# Autodesk Inventor assembly: MAIN
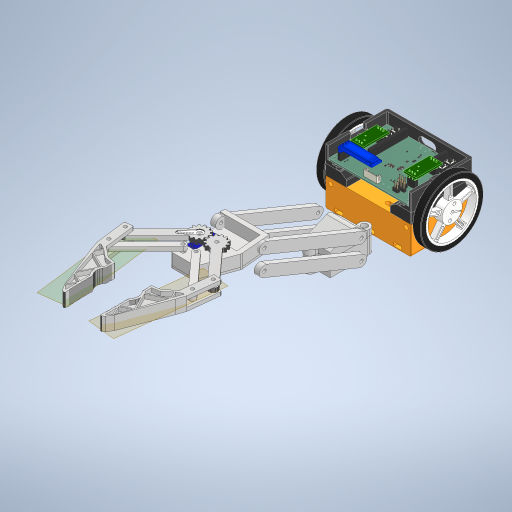
[picture p0: Inventor's stored thumbnail of the model, 512x512]
Saved by Autodesk Inventor 2023 (Build 270158000, 158)
## iProperties
Created: 2024-04-25
Part Number: MAIN
Document SubType Name: Assembly
Designer: Kamil
Author: Kamil
## Documents named in this file (24)
- C:\Users\kamil\Documents\PROJECTS - repos\ModBot---Projekt-Zespolowy\mechanics\MAIN.iam
- C:\Users\kamil\Documents\PROJECTS - repos\ModBot---Projekt-Zespolowy\mechanics\PololuWheel 60x8mm.ipt
- C:\Users\kamil\Documents\PROJECTS - repos\ModBot---Projekt-Zespolowy\mechanics\N20 DC MOTOR.ipt
- C:\Users\kamil\Documents\PROJECTS - repos\ModBot---Projekt-Zespolowy\mechanics\podst.ipt
- C:\Users\kamil\Documents\PROJECTS - repos\ModBot---Projekt-Zespolowy\mechanics\Li_Pol 800mAh.ipt
- C:\Users\kamil\Documents\PROJECTS - repos\ModBot---Projekt-Zespolowy\mechanics\pokrywka_baterii.ipt
- C:\Users\kamil\Documents\PROJECTS - repos\ModBot---Projekt-Zespolowy\mechanics\N20_Bracket_Extended_Pololu.ipt
- C:\Users\kamil\Documents\PROJECTS - repos\ModBot---Projekt-Zespolowy\mechanics\N20_Bracket_Extended_Pololu_MIR.ipt
- C:\Users\kamil\Documents\PROJECTS - repos\ModBot---Projekt-Zespolowy\mechanics\tyl.ipt
- C:\Users\kamil\Documents\PROJECTS - repos\ModBot---Projekt-Zespolowy\mechanics\podstawa_PCB.ipt
- C:\Users\kamil\Documents\PROJECTS - repos\ModBot---Projekt-Zespolowy\mechanics\pcb_glowne.ipt
- C:\Users\kamil\Documents\PROJECTS - repos\ModBot---Projekt-Zespolowy\mechanics\dach.ipt
- C:\Users\kamil\Documents\PROJECTS - repos\ModBot---Projekt-Zespolowy\mechanics\MS_podstawa.ipt
- C:\Users\kamil\Documents\PROJECTS - repos\ModBot---Projekt-Zespolowy\mechanics\TOF_VL53L0X (1).ipt
- C:\Users\kamil\Documents\PROJECTS - repos\ModBot---Projekt-Zespolowy\mechanics\MS_Pokrywa.ipt
- C:\Users\kamil\Documents\PROJECTS - repos\ModBot---Projekt-Zespolowy\mechanics\TOF_golpins.iam
- C:\Users\kamil\Documents\PROJECTS - repos\ModBot---Projekt-Zespolowy\mechanics\MS_PCB.ipt
- C:\Users\kamil\Documents\PROJECTS - repos\ModBot---Projekt-Zespolowy\mechanics\TOF_golpins_MIR.iam
- C:\Users\kamil\Documents\PROJECTS - repos\ModBot---Projekt-Zespolowy\mechanics\STEP\Płytka główna.ipt
- C:\Users\kamil\Documents\PROJECTS - repos\ModBot---Projekt-Zespolowy\mechanics\STEP\ESP32.ipt
- C:\Users\kamil\Documents\PROJECTS - repos\ModBot---Projekt-Zespolowy\mechanics\STEP\Sterowniki silników.ipt
- C:\Users\kamil\Documents\PROJECTS - repos\ModBot---Projekt-Zespolowy\mechanics\STEP\TFT Display 0.69_96x16.ipt
- C:\Users\kamil\Documents\PROJECTS - repos\ModBot---Projekt-Zespolowy\mechanics\modbot.ipt
- C:\Users\kamil\Documents\PROJECTS - repos\ModBot---Projekt-Zespolowy\mechanics\modul_chwytaka\chwytak.iam
## Components (29 placed, 23 different names)
1. PololuWheel 60x8mm:1 — Zestawiające:1, Kątowe:1, Zestawiające:2, Zestawiające:5, Zestawiające:6, Równoległe:2
2. N20 DC MOTOR:1 — Zestawiające:1, Kątowe:1, Zestawiające:2, Równoległe:1, Zestawiające:9, Zestawiające:18, Zestawiające:19
3. PololuWheel 60x8mm:2 — Zestawiające:5, Zestawiające:6, Zestawiające:10
4. N20 DC MOTOR:2 — Równoległe:1, Zestawiające:7
5. podst:1 — Zestawiające:9, Zestawiające:10, Zestawiające:11, Zestawiające:13, Równoległe:6, Zestawiające:14, Zestawiające:20, Zestawiające:33, Równoległe:22, Równoległe:23, Zestawiające:40, Zestawiające:50, Zestawiające:57, Równoległe:38
6. Li_Pol 800mAh:1 — Zestawiające:11, Zestawiające:13
7. pokrywka_baterii:1 — Równoległe:6, Zestawiające:14
8. N20_Bracket_Extended_Pololu:1 — Zestawiające:18, Zestawiające:19, Zestawiające:29, Zestawiające:69, Równoległe:37
9. N20_Bracket_Extended_Pololu_MIR:1 — Równoległe:17, Równoległe:18
10. tyl:1 — Zestawiające:20
11. podstawa_PCB:1 — Zestawiające:29, Równoległe:17, Równoległe:18, Zestawiające:30, Zestawiające:31, Równoległe:19, Równoległe:25, Zestawiające:61, Zestawiające:62, Zestawiające:63, Równoległe:35, Równoległe:36, Zestawiające:68, Zestawiające:70
12. pcb_glowne:1 — Zestawiające:30, Zestawiające:31, Równoległe:19
13. dach:1 — Równoległe:35, Równoległe:36, Zestawiające:68
14. MS_podstawa:1 — Zestawiające:33, Równoległe:22, Równoległe:23, Zestawiające:34, Zestawiające:35, Równoległe:24, Zestawiające:39, Zestawiające:43, Zestawiające:49, Zestawiające:51, Zestawiające:52, Zestawiające:56
15. TOF_VL53L0X (1):2 — Zestawiające:39, Zestawiające:40, Zestawiające:46
16. MS_Pokrywa:1 — Zestawiające:34, Zestawiające:35, Równoległe:24, Zestawiające:59
17. TOF_VL53L0X (1):4 — Zestawiające:43, Zestawiające:46
18. TOF_golpins:1 [sub-assembly] — Zestawiające:49, Zestawiające:50, Zestawiające:51, Zestawiające:54
19. TOF_golpins:2 [sub-assembly] — Zestawiające:52, Zestawiające:54, Zestawiające:58, Zestawiające:59
20. MS_PCB:1 — Zestawiające:56, Zestawiające:57, Zestawiające:58
21. TOF_golpins_MIR:1 [sub-assembly] — Zestawiające:60
22. TOF_golpins_MIR:2 [sub-assembly] — Zestawiające:60
23. Płytka główna:1 — Równoległe:25, Zestawiające:61, Zestawiające:62, Zestawiające:63, Równoległe:27, Równoległe:28, Zestawiające:64, Równoległe:29, Zestawiające:65, Równoległe:30, Zestawiające:66, Równoległe:31, Równoległe:32, Zestawiające:67, Równoległe:33, Równoległe:34
24. ESP32:1 — Równoległe:27, Równoległe:28, Zestawiające:64
25. Sterowniki silników:1 — Równoległe:29, Zestawiające:65, Równoległe:30
26. Sterowniki silników:2 — Zestawiające:66, Równoległe:31, Równoległe:32
27. TFT Display 0.69_96x16:1 — Zestawiające:67, Równoległe:33, Równoległe:34
28. modbot:1 — Zestawiające:69, Równoległe:37, Zestawiające:70
29. chwytak:1 [sub-assembly] — Równoległe:38
## Relationships (69: Mate 45, Flush 22, Angle 2)
- Zestawiające:1 [Mate]: PololuWheel 60x8mm:1 ↔ N20 DC MOTOR:1
- Kątowe:1 [Angle] (180 deg): PololuWheel 60x8mm:1 ↔ N20 DC MOTOR:1
- Zestawiające:2 [Mate]: PololuWheel 60x8mm:1 ↔ N20 DC MOTOR:1
- [Mate]: PololuWheel 60x8mm:2 ↔ N20 DC MOTOR:2
- [Angle] (180 deg): PololuWheel 60x8mm:2 ↔ N20 DC MOTOR:2
- [Mate]: PololuWheel 60x8mm:2 ↔ N20 DC MOTOR:2
- Zestawiające:5 [Mate]: PololuWheel 60x8mm:1 ↔ PololuWheel 60x8mm:2
- Równoległe:1 [Flush]: N20 DC MOTOR:1 ↔ N20 DC MOTOR:2
- Zestawiające:6 [Mate] (-100 mm): PololuWheel 60x8mm:1 ↔ PololuWheel 60x8mm:2
- Zestawiające:7 [Mate]: N20 DC MOTOR:2
- Równoległe:2 [Flush]: PololuWheel 60x8mm:1
- Zestawiające:9 [Mate]: N20 DC MOTOR:1 ↔ podst:1
- Zestawiające:10 [Mate] (1 mm): PololuWheel 60x8mm:2 ↔ podst:1
- Zestawiające:11 [Mate]: podst:1 ↔ Li_Pol 800mAh:1
- Zestawiające:13 [Mate] (6 mm): podst:1 ↔ Li_Pol 800mAh:1
- Równoległe:6 [Flush]: podst:1 ↔ pokrywka_baterii:1
- Zestawiające:14 [Mate]: podst:1 ↔ pokrywka_baterii:1
- Zestawiające:18 [Mate]: N20 DC MOTOR:1 ↔ N20_Bracket_Extended_Pololu:1
- Zestawiające:19 [Mate]: N20 DC MOTOR:1 ↔ N20_Bracket_Extended_Pololu:1
- Zestawiające:20 [Mate]: podst:1 ↔ tyl:1
- Zestawiające:29 [Mate]: N20_Bracket_Extended_Pololu:1 ↔ podstawa_PCB:1
- Równoległe:17 [Flush]: N20_Bracket_Extended_Pololu_MIR:1 ↔ podstawa_PCB:1
- Równoległe:18 [Flush]: N20_Bracket_Extended_Pololu_MIR:1 ↔ podstawa_PCB:1
- Zestawiające:30 [Mate]: podstawa_PCB:1 ↔ pcb_glowne:1
- Zestawiające:31 [Mate] (0.1 mm): podstawa_PCB:1 ↔ pcb_glowne:1
- Równoległe:19 [Flush]: podstawa_PCB:1 ↔ pcb_glowne:1
- Zestawiające:33 [Mate]: podst:1 ↔ MS_podstawa:1
- Równoległe:22 [Flush]: podst:1 ↔ MS_podstawa:1
- Równoległe:23 [Flush]: podst:1 ↔ MS_podstawa:1
- Zestawiające:34 [Mate]: MS_podstawa:1 ↔ MS_Pokrywa:1
- Zestawiające:35 [Mate]: MS_podstawa:1 ↔ MS_Pokrywa:1
- Równoległe:24 [Flush]: MS_podstawa:1 ↔ MS_Pokrywa:1
- Zestawiające:39 [Mate] (3.1 mm): MS_podstawa:1 ↔ TOF_VL53L0X (1):2
- Zestawiające:40 [Mate] (2 mm): podst:1 ↔ TOF_VL53L0X (1):2
- Zestawiające:43 [Mate] (3.1 mm): MS_podstawa:1 ↔ TOF_VL53L0X (1):4
- Zestawiające:46 [Mate] (12.5 mm): TOF_VL53L0X (1):2 ↔ TOF_VL53L0X (1):4
- Zestawiające:49 [Mate] (2.1 mm): MS_podstawa:1 ↔ TOF_golpins:1
- Zestawiające:50 [Mate] (3 mm): podst:1 ↔ TOF_golpins:1
- Zestawiające:51 [Mate] (1 mm): MS_podstawa:1 ↔ TOF_golpins:1
- Zestawiające:52 [Mate] (2.1 mm): MS_podstawa:1 ↔ TOF_golpins:2
- Zestawiające:54 [Mate] (14 mm): TOF_golpins:1 ↔ TOF_golpins:2
- Zestawiające:56 [Mate]: MS_podstawa:1 ↔ MS_PCB:1
- Zestawiające:57 [Mate]: podst:1 ↔ MS_PCB:1
- Zestawiające:58 [Mate]: TOF_golpins:2 ↔ MS_PCB:1
- Zestawiające:59 [Mate] (-1.5 mm): MS_Pokrywa:1 ↔ TOF_golpins:2
- Zestawiające:60 [Mate] (14 mm): TOF_golpins_MIR:1 ↔ TOF_golpins_MIR:2
- Równoległe:25 [Flush]: podstawa_PCB:1 ↔ Płytka główna:1
- Zestawiające:61 [Mate]: podstawa_PCB:1 ↔ Płytka główna:1
- Zestawiające:62 [Mate] (0.1 mm): podstawa_PCB:1 ↔ Płytka główna:1
- Zestawiające:63 [Mate]: podstawa_PCB:1 ↔ Płytka główna:1
- Równoległe:27 [Flush]: Płytka główna:1 ↔ ESP32:1
- Równoległe:28 [Flush]: Płytka główna:1 ↔ ESP32:1
- Zestawiające:64 [Mate]: Płytka główna:1 ↔ ESP32:1
- Równoległe:29 [Flush]: Płytka główna:1 ↔ Sterowniki silników:1
- Zestawiające:65 [Mate]: Płytka główna:1 ↔ Sterowniki silników:1
- Równoległe:30 [Flush]: Płytka główna:1 ↔ Sterowniki silników:1
- Zestawiające:66 [Mate]: Płytka główna:1 ↔ Sterowniki silników:2
- Równoległe:31 [Flush]: Płytka główna:1 ↔ Sterowniki silników:2
- Równoległe:32 [Flush]: Płytka główna:1 ↔ Sterowniki silników:2
- Zestawiające:67 [Mate]: Płytka główna:1 ↔ TFT Display 0.69_96x16:1
- Równoległe:33 [Flush]: Płytka główna:1 ↔ TFT Display 0.69_96x16:1
- Równoległe:34 [Flush]: Płytka główna:1 ↔ TFT Display 0.69_96x16:1
- Równoległe:35 [Flush]: podstawa_PCB:1 ↔ dach:1
- Równoległe:36 [Flush]: podstawa_PCB:1 ↔ dach:1
- Zestawiające:68 [Mate]: podstawa_PCB:1 ↔ dach:1
- Zestawiające:69 [Mate] (0.25 mm): N20_Bracket_Extended_Pololu:1 ↔ modbot:1
- Równoległe:37 [Flush]: N20_Bracket_Extended_Pololu:1 ↔ modbot:1
- Zestawiające:70 [Mate]: podstawa_PCB:1 ↔ modbot:1
- Równoległe:38 [Flush] (5 mm): podst:1 ↔ chwytak:1
## Named parameters: d3_d2 = 0 mm, d4_d0 = 0 mm, d5_d1 = 180 deg
